# Autodesk Inventor assembly: UBG-Dribblerhalter v2
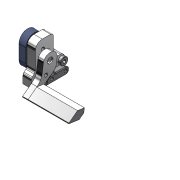
[picture p0: Inventor's stored thumbnail of the model, 180x180]
Saved by Autodesk Inventor 2022.3 (Build 263350000, 350)
## iProperties
Part Number: UBG-Dribblerhalter v2
Material: Generisch
Document SubType Name: Assembly
Designer: rYan
Mass: 41.0398 g
Surface Area: 116.754 cm^2
Volume: 13.2404 cm^3
Density: 3.09957 g/cm^3
Author: rYan
## Documents named in this file (18)
- D:\TIGERsGIT\Hardware\mechanik\2020\Inventor\Robot\Dribbler\UBG-Dribblerhalter v2.iam
- D:\TIGERsGIT\Hardware\mechanik\2020\Inventor\Inhaltscenter\de-DE\ISO 8745(2)\ISO 8745 - 4 x 10(6).ipt
- D:\TIGERsGIT\Hardware\mechanik\2020\Inventor\Purchased Parts\Zugfeder RZ-006DI.ipt
- D:\TIGERsGIT\Hardware\mechanik\2020\Inventor\Inhaltscenter\de-DE\DIN 7984\DIN 7984 - M3 x 5.ipt
- D:\TIGERsGIT\Hardware\mechanik\2020\Inventor\Purchased Parts\ISO 10642 - M3 x  6.ipt
- D:\TIGERsGIT\Hardware\mechanik\2020\Inventor\Robot\Dribbler\Dribbler Lagerbock v2.ipt
- D:\TIGERsGIT\Hardware\mechanik\2020\Inventor\Robot\Dribbler\Chipanschlag T0.5.ipt
- D:\TIGERsGIT\Hardware\mechanik\2020\Inventor\Robot\Dribbler\Chipanschlag T0.ipt
- D:\TIGERsGIT\Hardware\mechanik\2020\Inventor\Robot\Dribbler\Chipanschlag T1.ipt
- D:\TIGERsGIT\Hardware\mechanik\2020\Inventor\Inhaltscenter\de-DE\ISO 8745(2)\ISO 8745 - 2 x 10(6).ipt
- D:\TIGERsGIT\Hardware\mechanik\2020\Inventor\Robot\Kicker\MG-Chip Schaufel.iam
- D:\TIGERsGIT\Hardware\mechanik\2020\Inventor\Robot\Dribbler\Chipanschlag T1.5.ipt
- D:\TIGERsGIT\Hardware\mechanik\2020\Inventor\Robot\Dribbler\Chipanschlag T2.ipt
- D:\TIGERsGIT\Hardware\mechanik\2020\Inventor\Inhaltscenter\de-DE\ISO 10642(1)\ISO 10642 - M3 x  8.ipt
- D:\TIGERsGIT\Hardware\mechanik\2020\Inventor\Robot\Dribbler\Dribbler Slider.ipt
- D:\TIGERsGIT\Hardware\mechanik\2020\Inventor\Robot\Kicker\Chip Schaufel v2.ipt
- D:\TIGERsGIT\Hardware\mechanik\2020\Inventor\Robot\Dribbler\Chipanschlag TN1.ipt
- D:\TIGERsGIT\Hardware\mechanik\2020\Inventor\Robot\Dribbler\Chipanschlag TN2.ipt
## Components (25 placed, 17 different names)
1. Dribbler Lagerbock v2:3 — Passend:2, Passend:4, Symmetrie:1, Passend:5, Einfügen:4, Passend:6, Winkel:1, Einfügen:5, Einfügen:16, Passend:9, Einfügen:17, Passend:10, Einfügen:18, Passend:11, Einfügen:19, Einfügen:20, Einfügen:23, Passend:13, Einfügen:24, Passend:14, Einfügen:26, Passend:16, Einfügen:29, Winkel:2, Einfügen:30
2. Dribbler Lagerbock v2:4 — Passend:1, Passend:3, Symmetrie:1, Passend:5, Einfügen:3, Einfügen:6, Passend:12, Einfügen:25, Passend:15, Passend:17, Passend:18
3. DIN EN ISO 8745 4 x 10:3 — Einfügen:4
4. DIN EN ISO 8745 4 x 10:4 — Einfügen:3
5. Chip Schaufel v2:1 — Passend:6, Fluchtend:1, Winkel:1, Einfügen:9, Einfügen:10
6. Zugfeder RZ-006DI:1
7. DIN 7984 M3 x 5:1 — Einfügen:5
8. DIN 7984 M3 x 5:2 — Einfügen:6
9. ISO 10642 M3 x  6:1 — Einfügen:10
10. ISO 10642 M3 x  6:2 — Einfügen:9
11. Chipanschlag T0:1 — Einfügen:17, Passend:10
12. Chipanschlag T0.5:1 — Einfügen:16, Passend:9
13. Chipanschlag T1:1 — Einfügen:18, Passend:11
14. Chipanschlag T1.5:1 — Einfügen:23, Passend:13
15. Chipanschlag T2:1 — Einfügen:24, Passend:14
16. DIN EN ISO 8745 2 x 10:1 — Einfügen:19
17. DIN EN ISO 8745 2 x 10:2 — Einfügen:20, Passend:21, Passend:22
18. MG-Chip Schaufel:1 [sub-assembly] — Fluchtend:2, Passend:12, Winkel:2
19. ISO 10642 M3 x  8:1 — Einfügen:28
20. ISO 10642 M3 x  8:2 — Einfügen:27
21. Dribbler Slider:1 — Einfügen:26, Passend:16, Einfügen:28, Einfügen:31
22. Dribbler Slider:2 — Einfügen:25, Passend:15, Einfügen:27
23. Chipanschlag TN1:2 — Einfügen:29, Passend:21
24. Chipanschlag TN2:3 — Einfügen:30, Passend:22
25. ISO 10642 M3 x  8:3 — Einfügen:31
## Relationships (45: Mate 20, Insert 20, Flush 2, Angle 2, Symmetry 1)
- Passend:1 [Mate]: Dribbler Lagerbock v2:4
- Passend:2 [Mate]: Dribbler Lagerbock v2:3
- Passend:3 [Mate]: Dribbler Lagerbock v2:4
- Passend:4 [Mate]: Dribbler Lagerbock v2:3
- Symmetrie:1: Dribbler Lagerbock v2:3 ↔ Dribbler Lagerbock v2:4
- Passend:5 [Mate] (67.5 mm): Dribbler Lagerbock v2:3 ↔ Dribbler Lagerbock v2:4
- Einfügen:3 [Insert] (0.5 mm): Dribbler Lagerbock v2:4 ↔ DIN EN ISO 8745 4 x 10:4
- Einfügen:4 [Insert] (0.5 mm): Dribbler Lagerbock v2:3 ↔ DIN EN ISO 8745 4 x 10:3
- Passend:6 [Mate]: Dribbler Lagerbock v2:3 ↔ Chip Schaufel v2:1
- Fluchtend:1 [Flush]: Chip Schaufel v2:1
- Winkel:1 [Angle] (0 deg): Dribbler Lagerbock v2:3 ↔ Chip Schaufel v2:1
- Einfügen:5 [Insert] (1 mm): Dribbler Lagerbock v2:3 ↔ DIN 7984 M3 x 5:1
- Einfügen:6 [Insert] (1 mm): Dribbler Lagerbock v2:4 ↔ DIN 7984 M3 x 5:2
- Einfügen:9 [Insert]: Chip Schaufel v2:1 ↔ ISO 10642 M3 x  6:2
- Einfügen:10 [Insert]: Chip Schaufel v2:1 ↔ ISO 10642 M3 x  6:1
- Einfügen:16 [Insert]: Dribbler Lagerbock v2:3 ↔ Chipanschlag T0.5:1
- Passend:9 [Mate]: Dribbler Lagerbock v2:3 ↔ Chipanschlag T0.5:1
- Einfügen:17 [Insert]: Dribbler Lagerbock v2:3 ↔ Chipanschlag T0:1
- Passend:10 [Mate]: Dribbler Lagerbock v2:3 ↔ Chipanschlag T0:1
- Einfügen:18 [Insert]: Dribbler Lagerbock v2:3 ↔ Chipanschlag T1:1
- Passend:11 [Mate]: Dribbler Lagerbock v2:3 ↔ Chipanschlag T1:1
- Einfügen:19 [Insert]: Dribbler Lagerbock v2:3 ↔ DIN EN ISO 8745 2 x 10:1
- Einfügen:20 [Insert]: Dribbler Lagerbock v2:3 ↔ DIN EN ISO 8745 2 x 10:2
- Fluchtend:2 [Flush]: MG-Chip Schaufel:1
- Passend:12 [Mate]: Dribbler Lagerbock v2:4 ↔ MG-Chip Schaufel:1
- Einfügen:23 [Insert]: Dribbler Lagerbock v2:3 ↔ Chipanschlag T1.5:1
- Passend:13 [Mate]: Dribbler Lagerbock v2:3 ↔ Chipanschlag T1.5:1
- Einfügen:24 [Insert]: Dribbler Lagerbock v2:3 ↔ Chipanschlag T2:1
- Passend:14 [Mate]: Dribbler Lagerbock v2:3 ↔ Chipanschlag T2:1
- Einfügen:25 [Insert]: Dribbler Lagerbock v2:4 ↔ Dribbler Slider:2
- Passend:15 [Mate]: Dribbler Lagerbock v2:4 ↔ Dribbler Slider:2
- Einfügen:26 [Insert]: Dribbler Lagerbock v2:3 ↔ Dribbler Slider:1
- Passend:16 [Mate]: Dribbler Lagerbock v2:3 ↔ Dribbler Slider:1
- Einfügen:27 [Insert]: ISO 10642 M3 x  8:2 ↔ Dribbler Slider:2
- Einfügen:28 [Insert]: ISO 10642 M3 x  8:1 ↔ Dribbler Slider:1
- Passend:17 [Mate]: Dribbler Lagerbock v2:4
- Passend:18 [Mate]: Dribbler Lagerbock v2:4
- Passend:19 [Mate]
- Passend:20 [Mate]
- Einfügen:29 [Insert]: Dribbler Lagerbock v2:3 ↔ Chipanschlag TN1:2
- Passend:21 [Mate]: DIN EN ISO 8745 2 x 10:2 ↔ Chipanschlag TN1:2
- Winkel:2 [Angle] (8 deg): Dribbler Lagerbock v2:3 ↔ MG-Chip Schaufel:1
- Einfügen:30 [Insert]: Dribbler Lagerbock v2:3 ↔ Chipanschlag TN2:3
- Passend:22 [Mate]: DIN EN ISO 8745 2 x 10:2 ↔ Chipanschlag TN2:3
- Einfügen:31 [Insert]: Dribbler Slider:1 ↔ ISO 10642 M3 x  8:3
